# Autodesk Inventor assembly: Ensamble
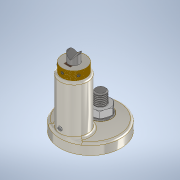
[picture p0: Inventor's stored thumbnail of the model, 180x180]
Saved by Autodesk Inventor 2020 (Build 240168000, 168)
## iProperties
Created: 2020-09-17
Part Number: Ensamble
Document SubType Name: Assembly
Designer: aaron
Author: aaron
## Documents named in this file (11)
- C:\Users\aaron\OneDrive\Escritorio\Tarea de especialidad\Ensamble.iam
- C:\Users\aaron\OneDrive\Escritorio\Tarea de especialidad\Base.ipt
- C:\Users\aaron\OneDrive\Escritorio\Tarea de especialidad\Arandela.ipt
- C:\Users\aaron\OneDrive\Escritorio\Tarea de especialidad\Perno de Sujeción.ipt
- C:\Users\aaron\OneDrive\Escritorio\Tarea de especialidad\Tca. Hex estandar.ipt
- C:\Users\aaron\OneDrive\Escritorio\Tarea de especialidad\Tornillo deslizante.ipt
- C:\Users\aaron\OneDrive\Escritorio\Tarea de especialidad\Tornillo de presion punta fuerte.ipt
- C:\Users\aaron\OneDrive\Escritorio\Tarea de especialidad\Tuerca moleteada.ipt
- C:\Users\aaron\OneDrive\Escritorio\Tarea de especialidad\Plaqueta Fosforbronce.ipt
- C:\Users\aaron\OneDrive\Escritorio\Tarea de especialidad\Rans10 punta plana.ipt
- C:\Users\aaron\OneDrive\Escritorio\Tarea de especialidad\Yunque V.ipt
## Components (12 placed, 10 different names)
1. Base:1 — Insert:1, Insert:2, Insert:4, Insert:5, Insert:9
2. Arandela:1 — Insert:1
3. Perno de Sujeción:1 — Insert:2, Insert:3
4. Tca. Hex estandar:1 — Insert:3
5. Tornillo deslizante:1 — Insert:4
6. Tornillo de presion punta fuerte:1 — Insert:5
7. Tuerca moleteada:1 — Mate:1, Mate:2, Flush:1, Insert:6, Insert:7, Insert:8, Insert:9, Insert:10
8. Plaqueta Fosforbronce:1 — Mate:1, Mate:2, Flush:1
9. Rans10 punta plana:1 — Insert:6
10. Rans10 punta plana:2 — Insert:7
11. Rans10 punta plana:3 — Insert:8
12. Yunque V:1 — Insert:10
## Relationships (13: Insert 10, Mate 2, Flush 1)
- Insert:1: Base:1 ↔ Arandela:1
- Insert:2: Base:1 ↔ Perno de Sujeción:1
- Insert:3: Perno de Sujeción:1 ↔ Tca. Hex estandar:1
- Insert:4: Base:1 ↔ Tornillo deslizante:1
- Insert:5: Base:1 ↔ Tornillo de presion punta fuerte:1
- Mate:1: Tuerca moleteada:1 ↔ Plaqueta Fosforbronce:1
- Mate:2: Tuerca moleteada:1 ↔ Plaqueta Fosforbronce:1
- Flush:1: Tuerca moleteada:1 ↔ Plaqueta Fosforbronce:1
- Insert:6: Tuerca moleteada:1 ↔ Rans10 punta plana:1
- Insert:7: Tuerca moleteada:1 ↔ Rans10 punta plana:2
- Insert:8 (-11 mm): Tuerca moleteada:1 ↔ Rans10 punta plana:3
- Insert:9: Base:1 ↔ Tuerca moleteada:1
- Insert:10: Tuerca moleteada:1 ↔ Yunque V:1
